# Autodesk Inventor assembly: R-I v7
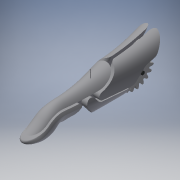
[picture p0: Inventor's stored thumbnail of the model, 180x180]
Saved by Autodesk Inventor 2018 (Build 220112000, 112)
## iProperties
Created: 2017-09-22
Part Number: R-I v7
Material: 一般
Document SubType Name: Assembly
Designer: sktom
Author: sktom
## Documents named in this file (12)
- D:\cloudstrage\NextCloud\Cad_mechanical\HACKberry_SizeM\3Dmodel\R\M-R-H\M-R-I\M-R-I .iam
- D:\cloudstrage\NextCloud\Cad_mechanical\HACKberry_SizeM\3Dmodel\R\M-R-H\M-R-I\M-R-I-other1.ipt
- D:\cloudstrage\NextCloud\Cad_mechanical\HACKberry_SizeM\3Dmodel\R\M-R-H\M-R-I\M-R-I-01.ipt
- D:\cloudstrage\NextCloud\Cad_mechanical\HACKberry_SizeM\3Dmodel\R\M-R-H\M-R-I\M-R-I-02.ipt
- D:\cloudstrage\NextCloud\Cad_mechanical\HACKberry_SizeM\3Dmodel\R\M-R-H\M-R-I\M-R-I-04.ipt
- D:\cloudstrage\NextCloud\Cad_mechanical\HACKberry_SizeM\3Dmodel\R\M-R-H\M-R-I\M-R-I-05.ipt
- D:\cloudstrage\NextCloud\Cad_mechanical\HACKberry_SizeM\3Dmodel\R\M-R-H\M-R-I\M-R-I-06.ipt
- D:\cloudstrage\NextCloud\Cad_mechanical\HACKberry_SizeM\3Dmodel\R\M-R-H\M-R-I\M-R-I-07.ipt
- D:\cloudstrage\NextCloud\Cad_mechanical\HACKberry_SizeM\3Dmodel\R\M-R-H\M-R-I\TOS 0.ipt
- D:\cloudstrage\NextCloud\Cad_mechanical\HACKberry_SizeM\3Dmodel\R\M-R-H\M-R-I\M1.7_L8.ipt
- D:\cloudstrage\NextCloud\Cad_mechanical\HACKberry_SizeM\3Dmodel\R\M-R-H\M-R-I\Shaft_phi2_L12.ipt
- D:\cloudstrage\NextCloud\Cad_mechanical\HACKberry_SizeM\3Dmodel\R\M-R-H\M-R-I\M-R-I-03.ipt
## Components (14 placed, 11 different names)
1. R-I-other1 v1:1 — 円柱状:1, 円柱状:2, 円柱状:3, 円柱状:4, 回転:8
2. R-I-01 v1:1 — 円柱状:1, 円柱状:2, 回転:2, 挿入:5
3. R-I-02 v1:1 — 回転:2, 回転:3, 回転:4, 円柱状:3, 挿入:3, 挿入:4
4. R-I-04 v1:1 — 回転:3, 回転:4
5. R-I-05 v1:1
6. R-I-06 v1:1 — 回転:5, 回転:6, 円柱状:4, 挿入:1, 挿入:2
7. R-I-07 v1:1 — 回転:5, 回転:6
8. TOS 0 v1:1 — 挿入:5
9. M1.7_L8:1 — 挿入:1
10. M1.7_L8:2 — 挿入:2
11. M1.7_L8:3 — 挿入:3
12. M1.7_L8:4 — 挿入:4
13. Shaft_phi2_L12:1 — 回転:8, 円柱状:5
14. 平歯車2:1 — 円柱状:5
## Relationships (16: RevoluteJoint 6, CylindricalJoint 5, Insert 5)
- 円柱状:1 [CylindricalJoint]: R-I-other1 v1:1 ↔ R-I-01 v1:1
- 円柱状:2 [CylindricalJoint]: R-I-other1 v1:1 ↔ R-I-01 v1:1
- 回転:2 [RevoluteJoint] (0.2 mm): R-I-01 v1:1 ↔ R-I-02 v1:1
- 回転:3 [RevoluteJoint]: R-I-02 v1:1 ↔ R-I-04 v1:1
- 回転:4 [RevoluteJoint]: R-I-02 v1:1 ↔ R-I-04 v1:1
- 回転:5 [RevoluteJoint]: R-I-06 v1:1 ↔ R-I-07 v1:1
- 回転:6 [RevoluteJoint]: R-I-06 v1:1 ↔ R-I-07 v1:1
- 円柱状:3 [CylindricalJoint]: R-I-other1 v1:1 ↔ R-I-02 v1:1
- 円柱状:4 [CylindricalJoint]: R-I-other1 v1:1 ↔ R-I-06 v1:1
- 挿入:1 [Insert]: R-I-06 v1:1 ↔ M1.7_L8:1
- 挿入:2 [Insert]: R-I-06 v1:1 ↔ M1.7_L8:2
- 挿入:3 [Insert]: R-I-02 v1:1 ↔ M1.7_L8:3
- 挿入:4 [Insert]: R-I-02 v1:1 ↔ M1.7_L8:4
- 挿入:5 [Insert]: R-I-01 v1:1 ↔ TOS 0 v1:1
- 回転:8 [RevoluteJoint]: R-I-other1 v1:1 ↔ Shaft_phi2_L12:1
- 円柱状:5 [CylindricalJoint]: Shaft_phi2_L12:1 ↔ 平歯車2:1
